# Autodesk Inventor assembly: ConeAssembly
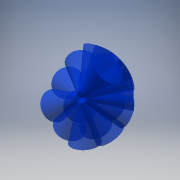
[picture p0: Inventor's stored thumbnail of the model, 180x180]
Saved by Autodesk Inventor 2019 (Build 230136000, 136)
## iProperties
Created: 2019-08-21
Part Number: ConeAssembly
Document SubType Name: Assembly
Designer: Dean
Author: Dean
## Documents named in this file (2)
- C:\Users\Dean\Documents\GitHub\AFRL2019\ConeAssembly.iam
- C:\Users\Dean\Documents\GitHub\AFRL2019\cone.ipt
## Components (19 placed, 1 different names)
1. cone:1 — Angle:2, Angle:3, Tangent:1, Tangent:5, Angle:15, Tangent:16, Angle:19, Tangent:20, Angle:22, Tangent:23
2. cone:2 — Angle:1, Angle:2, Tangent:1, Tangent:2, Angle:5, Tangent:3, Angle:7, Tangent:6, Tangent:15
3. cone:3 — Angle:1, Angle:3, Tangent:2, Angle:4, Tangent:4, Tangent:5
4. cone:4 — Angle:4, Angle:5, Tangent:3, Tangent:4, Angle:6, Tangent:7, Angle:8, Tangent:8
5. cone:5 — Angle:6, Angle:7, Tangent:6, Tangent:7, Angle:9, Tangent:9, Angle:11, Tangent:10, Angle:12, Tangent:12
6. cone:6 — Angle:8, Angle:9, Tangent:8, Tangent:9, Angle:10, Tangent:11
7. cone:7 — Angle:10, Angle:11, Tangent:10, Tangent:11, Angle:13, Tangent:13, Angle:29, Tangent:30
8. cone:8 — Angle:14, Tangent:14, Tangent:15, Angle:16, Tangent:17, Angle:18, Tangent:19
9. cone:9 — Angle:15, Tangent:16, Angle:16, Tangent:17, Angle:17, Tangent:18, Angle:20, Tangent:21, Angle:28, Tangent:29
10. cone:10 — Angle:12, Angle:13, Tangent:12, Tangent:13, Angle:14, Tangent:14, Angle:30, Tangent:31, Angle:32, Tangent:33
11. cone:11 — Angle:17, Angle:18, Tangent:18, Tangent:19, Angle:27, Tangent:28
12. cone:12 — Angle:19, Angle:20, Tangent:20, Tangent:21, Angle:21, Tangent:22, Angle:23, Tangent:24, Angle:26, Tangent:26
13. cone:13 — Angle:21, Angle:22, Tangent:22, Tangent:23, Angle:24, Tangent:25
14. cone:14 — Angle:27, Angle:28, Tangent:28, Tangent:29
15. cone:15 — Angle:25, Angle:26, Tangent:26, Tangent:27, Angle:33, Tangent:35
16. cone:16 — Angle:23, Angle:24, Tangent:24, Tangent:25, Angle:25, Tangent:27, Angle:34, Tangent:34
17. cone:17 — Angle:31, Angle:32, Tangent:32, Tangent:33
18. cone:18 — Angle:29, Angle:30, Tangent:30, Tangent:31, Angle:31, Tangent:32
19. cone:20 — Angle:33, Angle:34, Tangent:34, Tangent:35
## Relationships (69: Tangent 35, Angle 34)
- Angle:1 (30 deg): cone:2 ↔ cone:3
- Angle:2 (30 deg): cone:1 ↔ cone:2
- Angle:3 (30 deg): cone:1 ↔ cone:3
- Tangent:1: cone:1 ↔ cone:2
- Tangent:2: cone:2 ↔ cone:3
- Angle:4 (30 deg): cone:3 ↔ cone:4
- Angle:5 (30 deg): cone:2 ↔ cone:4
- Tangent:3: cone:2 ↔ cone:4
- Tangent:4: cone:3 ↔ cone:4
- Tangent:5: cone:1 ↔ cone:3
- Angle:6 (-30 deg): cone:4 ↔ cone:5
- Angle:7 (30 deg): cone:2 ↔ cone:5
- Tangent:6: cone:2 ↔ cone:5
- Tangent:7: cone:4 ↔ cone:5
- Angle:8 (-30 deg): cone:4 ↔ cone:6
- Angle:9 (-30 deg): cone:5 ↔ cone:6
- Tangent:8: cone:4 ↔ cone:6
- Tangent:9: cone:5 ↔ cone:6
- Angle:10 (30 deg): cone:6 ↔ cone:7
- Angle:11 (30 deg): cone:5 ↔ cone:7
- Tangent:10: cone:5 ↔ cone:7
- Tangent:11: cone:6 ↔ cone:7
- Angle:12 (30 deg): cone:5 ↔ cone:10
- Angle:13 (-30 deg): cone:7 ↔ cone:10
- Tangent:12: cone:5 ↔ cone:10
- Tangent:13: cone:7 ↔ cone:10
- Angle:14 (-30 deg): cone:8 ↔ cone:10
- Tangent:14: cone:8 ↔ cone:10
- Tangent:15: cone:2 ↔ cone:8
- Angle:15 (-30 deg): cone:1 ↔ cone:9
- Tangent:16: cone:1 ↔ cone:9
- Angle:16 (30 deg): cone:8 ↔ cone:9
- Tangent:17: cone:8 ↔ cone:9
- Angle:17 (-30 deg): cone:9 ↔ cone:11
- Angle:18 (-30 deg): cone:8 ↔ cone:11
- Tangent:18: cone:9 ↔ cone:11
- Tangent:19: cone:8 ↔ cone:11
- Angle:19 (-30 deg): cone:1 ↔ cone:12
- Angle:20 (-30 deg): cone:9 ↔ cone:12
- Tangent:20: cone:1 ↔ cone:12
- Tangent:21: cone:9 ↔ cone:12
- Angle:21 (-30 deg): cone:12 ↔ cone:13
- Angle:22 (30 deg): cone:1 ↔ cone:13
- Tangent:22: cone:12 ↔ cone:13
- Tangent:23: cone:1 ↔ cone:13
- Angle:23 (30 deg): cone:12 ↔ cone:16
- Angle:24 (30 deg): cone:13 ↔ cone:16
- Tangent:24: cone:12 ↔ cone:16
- Tangent:25: cone:13 ↔ cone:16
- Angle:25 (30 deg): cone:15 ↔ cone:16
- Angle:26 (30 deg): cone:12 ↔ cone:15
- Tangent:26: cone:12 ↔ cone:15
- Tangent:27: cone:15 ↔ cone:16
- Angle:27 (-30 deg): cone:11 ↔ cone:14
- Angle:28 (-30 deg): cone:9 ↔ cone:14
- Tangent:28: cone:11 ↔ cone:14
- Tangent:29: cone:9 ↔ cone:14
- Angle:29 (30 deg): cone:7 ↔ cone:18
- Angle:30 (-30 deg): cone:10 ↔ cone:18
- Tangent:30: cone:7 ↔ cone:18
- Tangent:31: cone:10 ↔ cone:18
- Angle:31 (-30 deg): cone:17 ↔ cone:18
- Angle:32 (-30 deg): cone:10 ↔ cone:17
- Tangent:32: cone:17 ↔ cone:18
- Tangent:33: cone:10 ↔ cone:17
- Angle:33 (-30 deg): cone:15 ↔ cone:20
- Angle:34 (30 deg): cone:16 ↔ cone:20
- Tangent:34: cone:16 ↔ cone:20
- Tangent:35: cone:15 ↔ cone:20
